# Autodesk Inventor assembly: Bar_connection_assembly
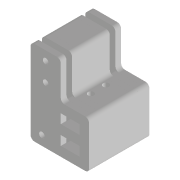
[picture p0: Inventor's stored thumbnail of the model, 180x180]
Saved by Autodesk Inventor 2022 (Build 260153000, 153)
## iProperties
Created: 2022-08-24
Part Number: Bar_connection_assembly
Document SubType Name: Assembly
Designer: dell
Author: dell
## Documents named in this file (4)
- D:\xxxx\Uni\Part IV\MECHENG_700\Part_IV_project_CAD\Bird_skeleton_prototypes\Wing_drone_V1\Bird_wing_V2\Wing_shoulder\Bar_connection_assembly.iam
- D:\xxxx\Uni\Part IV\MECHENG_700\Part_IV_project_CAD\Bird_skeleton_prototypes\Wing_drone_V1\Bird_wing_V2\Wing_shoulder\Bar_connection_plate.ipt
- D:\xxxx\Uni\Part IV\MECHENG_700\Part_IV_project_CAD\Bird_skeleton_prototypes\Wing_drone_V1\Bird_wing_V2\Wing_shoulder\Bar_connection_block.ipt
- D:\xxxx\Uni\Part IV\MECHENG_700\Part_IV_project_CAD\Bird_skeleton_prototypes\Wing_drone_V1\Bird_wing_V2\Wing_shoulder\Bar_connection_spacer.ipt
## Components (7 placed, 3 different names)
1. Bar_connection_plate:1
2. Bar_connection_block:1
3. Bar_connection_plate:2
4. Bar_connection_plate:3
5. Bar_connection_plate:4
6. Bar_connection_spacer:1
7. Bar_connection_spacer:2
## Relationships (18: Flush 12, Mate 6)
- [Mate]: Bar_connection_plate:1 ↔ Bar_connection_block:1
- [Flush]: Bar_connection_plate:1 ↔ Bar_connection_block:1
- [Flush]: Bar_connection_plate:1 ↔ Bar_connection_block:1
- [Mate]: Bar_connection_block:1 ↔ Bar_connection_plate:2
- [Flush]: Bar_connection_block:1 ↔ Bar_connection_plate:2
- [Flush]: Bar_connection_block:1 ↔ Bar_connection_plate:2
- [Mate] (3 mm): Bar_connection_plate:1 ↔ Bar_connection_plate:3
- [Flush]: Bar_connection_block:1 ↔ Bar_connection_plate:3
- [Flush]: Bar_connection_block:1 ↔ Bar_connection_plate:3
- [Mate] (3 mm): Bar_connection_plate:2 ↔ Bar_connection_plate:4
- [Flush]: Bar_connection_plate:2 ↔ Bar_connection_plate:4
- [Flush]: Bar_connection_plate:2 ↔ Bar_connection_plate:4
- [Mate]: Bar_connection_plate:1 ↔ Bar_connection_spacer:1
- [Flush]: Bar_connection_plate:3 ↔ Bar_connection_spacer:1
- [Flush]: Bar_connection_plate:3 ↔ Bar_connection_spacer:1
- [Mate]: Bar_connection_plate:2 ↔ Bar_connection_spacer:2
- [Flush]: Bar_connection_plate:4 ↔ Bar_connection_spacer:2
- [Flush]: Bar_connection_plate:4 ↔ Bar_connection_spacer:2
## Named parameters: d9_d15 = 0 mm, d10_d16 = 0 mm, d11_d17 = 0 mm
